# Autodesk Inventor assembly: BedActual
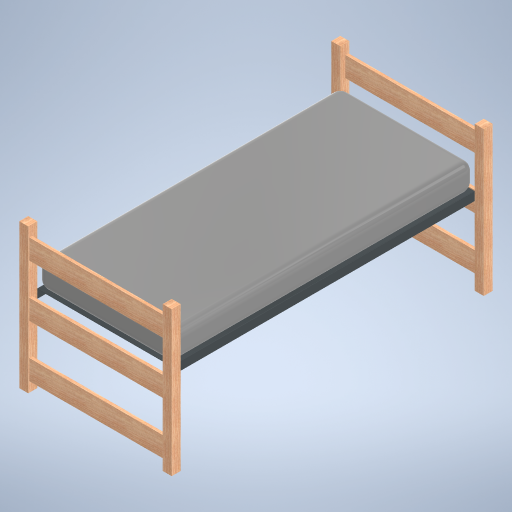
[picture p0: Inventor's stored thumbnail of the model, 512x512]
Saved by Autodesk Inventor 2023 (Build 270158000, 158)
## iProperties
Created: 2022-10-13
Part Number: BedActual
Document SubType Name: Assembly
Designer: mliu-23
Author: mliu-23
## Documents named in this file (4)
- D:\MyProfile\Documents\GitHub\VirtualPeddie\Furniture\CommonObj\CommonObj_Universal\(Bed Actual) CommonObj_Universal_BedActual\BedActual.iam
- D:\MyProfile\Documents\GitHub\VirtualPeddie\Furniture\CommonObj\CommonObj_Universal\(Bed Actual) CommonObj_Universal_BedActual\IronFrame.ipt
- D:\MyProfile\Documents\GitHub\VirtualPeddie\Furniture\CommonObj\CommonObj_Universal\(Bed Actual) CommonObj_Universal_BedActual\Matress.ipt
- D:\MyProfile\Documents\GitHub\VirtualPeddie\Furniture\CommonObj\CommonObj_Universal\(Bed Actual) CommonObj_Universal_BedActual\WoodFrame.ipt
## Components (4 placed, 3 different names)
1. IronFrame:1 — Mate:1, Flush:1, Flush:2
2. Matress:1 — Mate:1, Flush:1, Flush:2, Mate:3, Flush:3, Flush:4, Mate:4, Flush:5, Flush:6
3. WoodFrame:1 — Mate:3, Flush:3, Flush:4
4. WoodFrame:2 — Mate:4, Flush:5, Flush:6
## Relationships (9: Flush 6, Mate 3)
- Mate:1: IronFrame:1 ↔ Matress:1
- Flush:1: IronFrame:1 ↔ Matress:1
- Flush:2: IronFrame:1 ↔ Matress:1
- Mate:3: Matress:1 ↔ WoodFrame:1
- Flush:3 (-57.15 mm): Matress:1 ↔ WoodFrame:1
- Flush:4 (-203.2 mm): Matress:1 ↔ WoodFrame:1
- Mate:4: Matress:1 ↔ WoodFrame:2
- Flush:5 (-57.15 mm): Matress:1 ↔ WoodFrame:2
- Flush:6 (-203.2 mm): Matress:1 ↔ WoodFrame:2
